# Autodesk Inventor assembly: SLAVE ARM_exploded
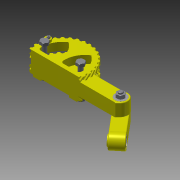
[picture p0: Inventor's stored thumbnail of the model, 180x180]
Saved by Autodesk Inventor 2014 (Build 180170000, 170)
## iProperties
Created: 2013-11-27
Part Number: SLAVE ARM_exploded
Document SubType Name: Assembly
Designer: employee
Author: employee
## Documents named in this file (8)
- C:\Dev\Work\Drukarka\ConceptFORGE\GUS Simpson\INVENTOR FILES\exploded_view\SLAVE ARM_exploded.iam
- C:\Dev\Work\Drukarka\ConceptFORGE\GUS Simpson\INVENTOR FILES\SLAVE ARM.ipt
- C:\Dev\Work\Drukarka\ConceptFORGE\GUS Simpson\INVENTOR FILES\ECCENTRIC STOP.ipt
- C:\Dev\Work\Drukarka\ConceptFORGE\GUS Simpson\INVENTOR FILES\M3x20.ipt
- C:\Dev\Work\Drukarka\ConceptFORGE\GUS Simpson\INVENTOR FILES\M8 NUT.ipt
- C:\Dev\Work\Drukarka\ConceptFORGE\GUS Simpson\INVENTOR FILES\_608.ipt
- C:\Dev\Work\Drukarka\ConceptFORGE\GUS Simpson\INVENTOR FILES\M8x60.ipt
- C:\Dev\Work\Drukarka\ConceptFORGE\GUS Simpson\INVENTOR FILES\HUB CENTER.iam
## Components (12 placed, 7 different names)
1. SLAVE ARM:1 — Insert:1, Insert:3, Insert:4, Insert:5, Insert:6, Insert:7, Insert:8, Angle:1, Angle:2, Angle:3, Angle:4, Angle:5, Angle:6, Angle:7
2. ECCENTRIC STOP:1 — Insert:1, Insert:2
3. M3x20:1 — Insert:2
4. M8 NUT:1 — Insert:5, Angle:3, Insert:9
5. M8 NUT:2 — Insert:7, Angle:2
6. M8 NUT:3 — Insert:6, Angle:4, Insert:10
7. M8 NUT:4 — Insert:8, Angle:1
8. _608:1 — Insert:4, Insert:11
9. _608:2 — Insert:3
10. Hex Bolt - Metric M8 x 1.25 x 60:1 — Insert:10, Angle:5
11. Hex Bolt - Metric M8 x 1.25 x 60:2 — Insert:9, Angle:6
12. HUB CENTER:1 [sub-assembly] — Insert:11, Angle:7
## Relationships (18: Insert 11, Angle 7)
- Insert:1: SLAVE ARM:1 ↔ ECCENTRIC STOP:1
- Insert:2: ECCENTRIC STOP:1 ↔ M3x20:1
- Insert:3: SLAVE ARM:1 ↔ _608:2
- Insert:4: SLAVE ARM:1 ↔ _608:1
- Insert:5: SLAVE ARM:1 ↔ M8 NUT:1
- Insert:6: SLAVE ARM:1 ↔ M8 NUT:3
- Insert:7: SLAVE ARM:1 ↔ M8 NUT:2
- Insert:8: SLAVE ARM:1 ↔ M8 NUT:4
- Angle:1 (0 deg): SLAVE ARM:1 ↔ M8 NUT:4
- Angle:2 (0 deg): SLAVE ARM:1 ↔ M8 NUT:2
- Angle:3 (0 deg): SLAVE ARM:1 ↔ M8 NUT:1
- Angle:4 (0 deg): SLAVE ARM:1 ↔ M8 NUT:3
- Insert:9 (-2 mm): M8 NUT:1 ↔ Hex Bolt - Metric M8 x 1.25 x 60:2
- Insert:10 (-2 mm): M8 NUT:3 ↔ Hex Bolt - Metric M8 x 1.25 x 60:1
- Angle:5 (0 deg): SLAVE ARM:1 ↔ Hex Bolt - Metric M8 x 1.25 x 60:1
- Angle:6 (0 deg): SLAVE ARM:1 ↔ Hex Bolt - Metric M8 x 1.25 x 60:2
- Insert:11: _608:1 ↔ HUB CENTER:1
- Angle:7 (-50 deg): SLAVE ARM:1 ↔ HUB CENTER:1
